# Autodesk Inventor assembly: Head
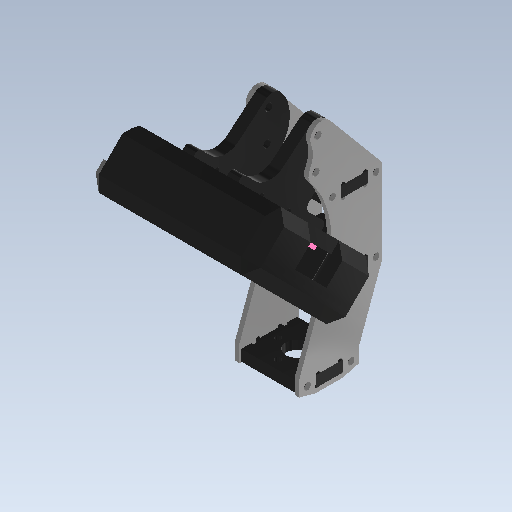
[picture p0: Inventor's stored thumbnail of the model, 512x512]
Saved by Autodesk Inventor 2020.4 (Build 244396000, 396)
## iProperties
Created: 2021-09-05
Part Number: Head
Document SubType Name: Assembly
Designer: Masato
Mass: 131.819 g
Surface Area: 530.417 cm^2
Volume: 94.4592 cm^3
Density: 1.39551 g/cm^3
Author: Masato
## Documents named in this file (8)
- C:\Users\masato\Documents\Inventor\CITBrains\OpenPlatform_ver3_0\UpperBody\Head\Head.iam
- C:\Users\masato\Documents\Inventor\CITBrains\OpenPlatform_ver3_0\Ready_Made\KBCR-S02MU.ipt
- C:\Users\masato\Documents\Inventor\CITBrains\OpenPlatform_ver3_0\UpperBody\Head\Camera_vertical_frame_01.ipt
- C:\Users\masato\Documents\Inventor\CITBrains\OpenPlatform_ver3_0\UpperBody\Head\Camera_horizontal_frame_01.ipt
- C:\Users\masato\Documents\Inventor\CITBrains\OpenPlatform_ver3_0\UpperBody\Head\Camera_cover_01.ipt
- C:\Users\masato\Documents\Inventor\CITBrains\OpenPlatform_ver3_0\UpperBody\Head\Head_horizontal_frame_01.ipt
- C:\Users\masato\Documents\Inventor\CITBrains\OpenPlatform_ver3_0\UpperBody\Head\Head_horizontal_frame_02.ipt
- C:\Users\masato\Documents\Inventor\CITBrains\OpenPlatform_ver3_0\UpperBody\Head\Head_vertical_frame_01.ipt
## Components (10 placed, 7 different names)
1. KBCR-S02MU:1 — 挿入:23, 挿入:24, 挿入:25, 挿入:26
2. Camera_vertical_frame_01:1 — 挿入:3, 挿入:7, 挿入:8, 挿入:33
3. Camera_vertical_frame_01:2 — 挿入:5, 挿入:6, 挿入:9, 挿入:10
4. Camera_horizontal_frame_01:1 — 挿入:3, 挿入:5, 挿入:6, 挿入:23, 挿入:24, 挿入:25, 挿入:26, 挿入:27, 挿入:28, 挿入:33
5. Camera_cover_01:1 — 挿入:27, 挿入:28
6. Head_horizontal_frame_01:1 — 挿入:29, 挿入:30, 挿入:31, 挿入:32
7. Head_horizontal_frame_02:1 — 挿入:11, 挿入:12, 挿入:15, 挿入:16
8. Head_horizontal_frame_02:2 — 挿入:13, 挿入:14, 挿入:17, 挿入:18
9. Head_vertical_frame_01:1 — 挿入:7, 挿入:8, 挿入:11, 挿入:12, 挿入:13, 挿入:14, 挿入:29, 挿入:30
10. Head_vertical_frame_01:2 — 挿入:9, 挿入:10, 挿入:15, 挿入:16, 挿入:17, 挿入:18, 挿入:31, 挿入:32
## Relationships (26: Insert 26)
- 挿入:3 [Insert]: Camera_vertical_frame_01:1 ↔ Camera_horizontal_frame_01:1
- 挿入:5 [Insert]: Camera_vertical_frame_01:2 ↔ Camera_horizontal_frame_01:1
- 挿入:6 [Insert]: Camera_vertical_frame_01:2 ↔ Camera_horizontal_frame_01:1
- 挿入:7 [Insert]: Camera_vertical_frame_01:1 ↔ Head_vertical_frame_01:1
- 挿入:8 [Insert]: Camera_vertical_frame_01:1 ↔ Head_vertical_frame_01:1
- 挿入:9 [Insert]: Camera_vertical_frame_01:2 ↔ Head_vertical_frame_01:2
- 挿入:10 [Insert]: Camera_vertical_frame_01:2 ↔ Head_vertical_frame_01:2
- 挿入:11 [Insert]: Head_horizontal_frame_02:1 ↔ Head_vertical_frame_01:1
- 挿入:12 [Insert]: Head_horizontal_frame_02:1 ↔ Head_vertical_frame_01:1
- 挿入:13 [Insert]: Head_horizontal_frame_02:2 ↔ Head_vertical_frame_01:1
- 挿入:14 [Insert]: Head_horizontal_frame_02:2 ↔ Head_vertical_frame_01:1
- 挿入:15 [Insert]: Head_horizontal_frame_02:1 ↔ Head_vertical_frame_01:2
- 挿入:16 [Insert]: Head_horizontal_frame_02:1 ↔ Head_vertical_frame_01:2
- 挿入:17 [Insert]: Head_horizontal_frame_02:2 ↔ Head_vertical_frame_01:2
- 挿入:18 [Insert]: Head_horizontal_frame_02:2 ↔ Head_vertical_frame_01:2
- 挿入:23 [Insert]: KBCR-S02MU:1 ↔ Camera_horizontal_frame_01:1
- 挿入:24 [Insert]: KBCR-S02MU:1 ↔ Camera_horizontal_frame_01:1
- 挿入:25 [Insert]: KBCR-S02MU:1 ↔ Camera_horizontal_frame_01:1
- 挿入:26 [Insert]: KBCR-S02MU:1 ↔ Camera_horizontal_frame_01:1
- 挿入:27 [Insert]: Camera_horizontal_frame_01:1 ↔ Camera_cover_01:1
- 挿入:28 [Insert]: Camera_horizontal_frame_01:1 ↔ Camera_cover_01:1
- 挿入:29 [Insert]: Head_horizontal_frame_01:1 ↔ Head_vertical_frame_01:1
- 挿入:30 [Insert]: Head_horizontal_frame_01:1 ↔ Head_vertical_frame_01:1
- 挿入:31 [Insert]: Head_horizontal_frame_01:1 ↔ Head_vertical_frame_01:2
- 挿入:32 [Insert]: Head_horizontal_frame_01:1 ↔ Head_vertical_frame_01:2
- 挿入:33 [Insert]: Camera_vertical_frame_01:1 ↔ Camera_horizontal_frame_01:1
